# Autodesk Inventor assembly: motor_wheel
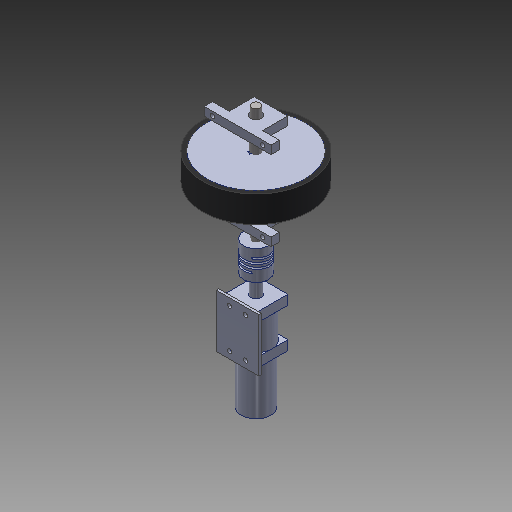
[picture p0: Inventor's stored thumbnail of the model, 512x512]
Saved by Autodesk Inventor 2018 (Build 220112000, 112)
## iProperties
Created: 2017-05-04
Part Number: motor_wheel
Document SubType Name: Assembly
Designer: AYUSH SHUKLA
Author: AYUSH SHUKLA
## Documents named in this file (9)
- C:\Study\BTP2\Robomuse Inventor CAD\motor_wheel\motor_wheel.iam
- C:\Study\BTP2\Robomuse Inventor CAD\motor_wheel\Drive_banebot_1_MIR.ipt
- C:\Study\BTP2\Robomuse Inventor CAD\motor_wheel\Drive_motor_mounting_1_MIR.ipt
- C:\Study\BTP2\Robomuse Inventor CAD\motor_wheel\Drive_helical_coupler_1_MIR.ipt
- C:\Study\BTP2\Robomuse Inventor CAD\motor_wheel\Wheel_core_1_MIR.ipt
- C:\Study\BTP2\Robomuse Inventor CAD\motor_wheel\Wheel_rubber_1_MIR.ipt
- C:\Study\BTP2\Robomuse Inventor CAD\motor_wheel\Drive_shaft_1_MIR.ipt
- C:\Study\BTP2\Robomuse Inventor CAD\motor_wheel\Drive_bearing_1_MIR.ipt
- C:\Study\BTP2\Robomuse Inventor CAD\motor_wheel\radial ball bearing_68_iso_ISO 15 RBB - 108 - 8,SI,NC,8_68_MIR.ipt
## Components (10 placed, 8 different names)
1. Drive_banebot_1_MIR:1 — Mate:18
2. Drive_motor_mounting_1_MIR:1 — Flush:3
3. Drive_helical_coupler_1_MIR:1 — Mate:18
4. Wheel_core_1_MIR:1 — Mate:17
5. Wheel_rubber_1_MIR:1
6. Drive_shaft_1_MIR:1
7. Drive_bearing_1_MIR:1 — Mate:17, Flush:2
8. radial ball bearing_68_iso_ISO 15 RBB - 108 - 8,SI,NC,8_68_MIR:1
9. Drive_bearing_1_MIR:2 — Mate:15, Mate:16, Flush:2, Flush:3
10. radial ball bearing_68_iso_ISO 15 RBB - 108 - 8,SI,NC,8_68_MIR:2 — Mate:15, Mate:16
## Relationships (21: Mate 18, Flush 3)
- [Mate]: Drive_banebot_1_MIR:1 ↔ Drive_motor_mounting_1_MIR:1
- [Mate]: Drive_banebot_1_MIR:1 ↔ Drive_motor_mounting_1_MIR:1
- [Mate]: Drive_banebot_1_MIR:1 ↔ Drive_motor_mounting_1_MIR:1
- [Mate]: Wheel_core_1_MIR:1 ↔ Wheel_rubber_1_MIR:1
- [Flush]: Wheel_core_1_MIR:1 ↔ Wheel_rubber_1_MIR:1
- [Mate]: Drive_banebot_1_MIR:1 ↔ Drive_shaft_1_MIR:1
- [Mate]: Wheel_core_1_MIR:1 ↔ Drive_shaft_1_MIR:1
- [Mate]: Drive_shaft_1_MIR:1 ↔ radial ball bearing_68_iso_ISO 15 RBB - 108 - 8,SI,NC,8_68_MIR:1
- [Mate]: Drive_bearing_1_MIR:1 ↔ radial ball bearing_68_iso_ISO 15 RBB - 108 - 8,SI,NC,8_68_MIR:1
- [Mate]: Drive_bearing_1_MIR:1 ↔ radial ball bearing_68_iso_ISO 15 RBB - 108 - 8,SI,NC,8_68_MIR:1
- [Mate]: Drive_shaft_1_MIR:1 ↔ Drive_bearing_1_MIR:2
- [Mate] (26.825 mm): Wheel_core_1_MIR:1 ↔ Drive_bearing_1_MIR:2
- [Mate] (9.9 mm): Drive_shaft_1_MIR:1 ↔ Drive_bearing_1_MIR:1
- [Mate]: Drive_helical_coupler_1_MIR:1 ↔ Drive_shaft_1_MIR:1
- [Mate] (22.5775 mm): Drive_helical_coupler_1_MIR:1 ↔ Drive_bearing_1_MIR:2
- Mate:15: Drive_bearing_1_MIR:2 ↔ radial ball bearing_68_iso_ISO 15 RBB - 108 - 8,SI,NC,8_68_MIR:2
- Mate:16: Drive_bearing_1_MIR:2 ↔ radial ball bearing_68_iso_ISO 15 RBB - 108 - 8,SI,NC,8_68_MIR:2
- Mate:17 (26.825 mm): Wheel_core_1_MIR:1 ↔ Drive_bearing_1_MIR:1
- Flush:2: Drive_bearing_1_MIR:1 ↔ Drive_bearing_1_MIR:2
- Mate:18 (22.5775 mm): Drive_banebot_1_MIR:1 ↔ Drive_helical_coupler_1_MIR:1
- Flush:3: Drive_motor_mounting_1_MIR:1 ↔ Drive_bearing_1_MIR:2
